# Autodesk Inventor assembly: Bearing
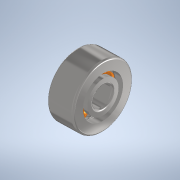
[picture p0: Inventor's stored thumbnail of the model, 180x180]
Saved by Autodesk Inventor 2020 (Build 240168000, 168)
## iProperties
Created: 2022-06-23
Part Number: Bearing
Document SubType Name: Assembly
Designer: karimi2
Author: karimi2
## Documents named in this file (4)
- C:\Users\karimi2\Documents\PROJECT\Bearing.iam
- C:\Users\karimi2\Documents\PROJECT\Ball Bearing\BearingPART1.ipt
- C:\Users\karimi2\Documents\PROJECT\Ball Bearing\BearingPART2.ipt
- C:\Users\karimi2\Documents\PROJECT\Ball Bearing\Ball.ipt
## Components (10 placed, 3 different names)
1. BearingPART1:1 — Mate:1, Flush:1, Tangent:1
2. BearingPART2:1 — Mate:1, Flush:1
3. Ball:1 — Tangent:1
4. Ball:2
5. Ball:3
6. Ball:4
7. Ball:5
8. Ball:6
9. Ball:7
10. Ball:8
## Component patterns: (8 elements, first: Ball:1)
## Relationships (3: Mate 1, Flush 1, Tangent 1)
- Mate:1: BearingPART1:1 ↔ BearingPART2:1
- Flush:1: BearingPART1:1 ↔ BearingPART2:1
- Tangent:1: BearingPART1:1 ↔ Ball:1
